# Autodesk Inventor assembly: GY81 Logger
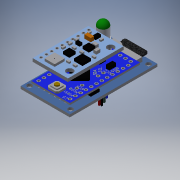
[picture p0: Inventor's stored thumbnail of the model, 180x180]
Saved by Autodesk Inventor 2016 (Build 200138000, 138)
## iProperties
Created: 2015-11-30
Part Number: GY81 Logger
Document SubType Name: Assembly
Designer: Spooner
Author: Spooner
## Documents named in this file (5)
- C:\Users\Spooner\Documents\GY81 Logger\3D Models\GY81 Logger.iam
- C:\Users\Spooner\Documents\GY81 Logger\3D Models\Arduino Pro Mini.ipt
- C:\Users\Spooner\Documents\GY81 Logger\3D Models\GY81.ipt
- C:\Users\Spooner\Documents\GY81 Logger\3D Models\MicroSD Card in Reader.iam
- C:\Users\Spooner\Documents\GY81 Logger\3D Models\Clipped LED.ipt
## Components (4 placed, 4 different names)
1. Arduino Pro Mini:1 — Flush:1, Flush:2, Mate:1, Mate:2
2. GY81:1 — Flush:3, Flush:4, Mate:2
3. MicroSD Card in Reader:1 [sub-assembly] — Flush:1, Flush:2, Mate:1, Flush:3, Flush:4, Mate:3, Flush:5, Flush:6
4. Clipped LED:1 — Mate:3, Flush:5, Flush:6
## Relationships (9: Flush 6, Mate 3)
- Flush:1: Arduino Pro Mini:1 ↔ MicroSD Card in Reader:1
- Flush:2: Arduino Pro Mini:1 ↔ MicroSD Card in Reader:1
- Mate:1 (3.81 mm): Arduino Pro Mini:1 ↔ MicroSD Card in Reader:1
- Flush:3: GY81:1 ↔ MicroSD Card in Reader:1
- Flush:4 (5.715 mm): GY81:1 ↔ MicroSD Card in Reader:1
- Mate:2 (2.54 mm): Arduino Pro Mini:1 ↔ GY81:1
- Mate:3 (2.54 mm): MicroSD Card in Reader:1 ↔ Clipped LED:1
- Flush:5 (3.81 mm): MicroSD Card in Reader:1 ↔ Clipped LED:1
- Flush:6 (3.175 mm): MicroSD Card in Reader:1 ↔ Clipped LED:1
